# Autodesk Inventor assembly: arm encoder
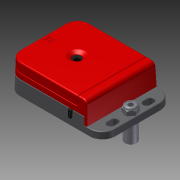
[picture p0: Inventor's stored thumbnail of the model, 180x180]
Saved by Autodesk Inventor 2014 SP1 (Build 180222100, 222)
## iProperties
Created: 2014-03-19
Part Number: arm encoder
Document SubType Name: Assembly
Designer: Ryan
Author: Ryan
## Documents named in this file (4)
- C:\Users\Ryan\Desktop\sw\toss up 4th robot\tower\arm encoder.iam
- C:\Users\Ryan\Desktop\sw\lib\Super Sonic Sparks VEX CAD Library\Motors & Sensors\Optical Shaft (Quadrature) Encoder.iam
- C:\Users\Ryan\Desktop\sw\lib\Aperture VEX CAD Library\Spacers\thin\SPACER-0320-0500.ipt
- C:\Users\Ryan\Desktop\sw\lib\Aperture VEX CAD Library\Hardware\8-32\8-32 nylock.ipt
## Components (3 placed, 3 different names)
1. Optical Shaft (Quadrature) Encoder:1 [sub-assembly] — Mate:1, Mate:2, Mate:4
2. SPACER-0320-0500:1 — Mate:1, Mate:2, Mate:3
3. 8-32 nylock:1 — Mate:3, Mate:4
## Relationships (4: Mate 4)
- Mate:1: Optical Shaft (Quadrature) Encoder:1 ↔ SPACER-0320-0500:1
- Mate:2: Optical Shaft (Quadrature) Encoder:1 ↔ SPACER-0320-0500:1
- Mate:3: SPACER-0320-0500:1 ↔ 8-32 nylock:1
- Mate:4: Optical Shaft (Quadrature) Encoder:1 ↔ 8-32 nylock:1
